# Autodesk Inventor assembly: ASM_Motor_Unit_Part2_Rev_disasm
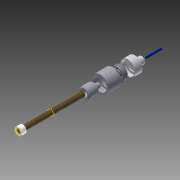
[picture p0: Inventor's stored thumbnail of the model, 180x180]
Saved by Autodesk Inventor 2011 SP2 (Build 150309200, 309)
## iProperties
Created: 2011-03-22
Part Number: ASM_Motor_Unit_Part2_Rev_disasm
Document SubType Name: Assembly
Designer: sungwook
Author: sungwook
## Documents named in this file (8)
- C:\Users\sungwook\Documents\Inventor\Micron20_Base_Tube_Adjst\Assembly\ASM_Motor_Unit_Part2_Rev_disasm.iam
- C:\Users\sungwook\Documents\Inventor\Micron20_Base_Tube_Adjst\Parts\Motor Units\MU_Motor_Thread.ipt
- C:\Users\sungwook\Documents\Inventor\Micron20_Base_Tube_Adjst\Parts\Motor Units\MU_Motor_Coupling_3.ipt
- C:\Users\sungwook\Documents\Inventor\Micron20_Base_Tube_Adjst\Parts\Motor Units\MU_Bearing_Housing_Inner.ipt
- C:\Users\sungwook\Documents\Inventor\Micron20_Base_Tube_Adjst\Parts\Motor Units\MU_Prolene.ipt
- C:\Users\sungwook\Documents\Inventor\Micron20_Base_Tube_Adjst\Parts\Motor Units\MU_Bearing(681h).ipt
- C:\Users\sungwook\Documents\Inventor\Micron20_Base_Tube_Adjst\Parts\Motor Units\MU_Bottom_Stop.ipt
- C:\Users\sungwook\Documents\Inventor\Micron20_Base_Tube_Adjst\Parts\Motor Units\MU_Bearing_Retainer.ipt
## Components (7 placed, 7 different names)
1. MU_Motor_Thread:1 — Mate:7, Flush:1, Mate:38, Flush:2
2. MU_Motor_Coupling_3:1 — Mate:7, Mate:22, Flush:1, Mate:27, Mate:28, Mate:40
3. MU_Bearing_Housing_Inner:1 — Mate:20, Mate:22, Mate:23, Mate:24, Mate:29, Mate:31
4. MU_Prolene:1 — Mate:20, Mate:23, Mate:24
5. MU_Bearing(681h):1 — Mate:27, Mate:28, Mate:29, Mate:31, Mate:39
6. MU_Bottom_Stop:1 — Mate:38, Flush:2
7. MU_Bearing_Retainer:1 — Mate:39, Mate:40
## Relationships (14: Mate 12, Flush 2)
- Mate:7: MU_Motor_Thread:1 ↔ MU_Motor_Coupling_3:1
- Mate:20: MU_Bearing_Housing_Inner:1 ↔ MU_Prolene:1
- Mate:22 (0.2 mm): MU_Motor_Coupling_3:1 ↔ MU_Bearing_Housing_Inner:1
- Mate:23: MU_Bearing_Housing_Inner:1 ↔ MU_Prolene:1
- Mate:24: MU_Bearing_Housing_Inner:1 ↔ MU_Prolene:1
- Flush:1: MU_Motor_Thread:1 ↔ MU_Motor_Coupling_3:1
- Mate:27: MU_Motor_Coupling_3:1 ↔ MU_Bearing(681h):1
- Mate:28: MU_Motor_Coupling_3:1 ↔ MU_Bearing(681h):1
- Mate:29: MU_Bearing_Housing_Inner:1 ↔ MU_Bearing(681h):1
- Mate:31: MU_Bearing_Housing_Inner:1 ↔ MU_Bearing(681h):1
- Mate:38: MU_Motor_Thread:1 ↔ MU_Bottom_Stop:1
- Flush:2: MU_Motor_Thread:1 ↔ MU_Bottom_Stop:1
- Mate:39: MU_Bearing(681h):1 ↔ MU_Bearing_Retainer:1
- Mate:40: MU_Motor_Coupling_3:1 ↔ MU_Bearing_Retainer:1
